# Autodesk Inventor assembly: B Idler
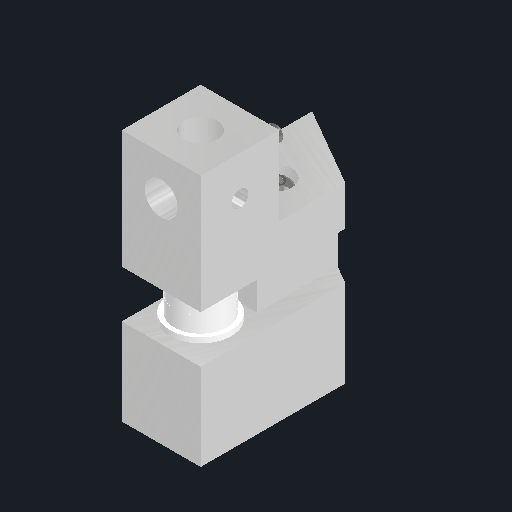
[picture p0: Inventor's stored thumbnail of the model, 512x512]
Saved by Autodesk Inventor 2025.1 (Build 291241020, 241B)
## iProperties
Created: 2025-05-09
Part Number: B Idler
Document SubType Name: Assembly
Designer: AdminForWorker
Title: B Idler
Author: AdminForWorker
## Documents named in this file (3)
- C:\Users\Joshua Eah\Documents\Voron 0.2\CAD\Master Assembly\B Idler.iam
- C:\Users\Joshua Eah\Documents\Voron 0.2\CAD\Master Assembly\Hardware\Hardware Assemblies\Hardware (10).iam
- C:\Users\Joshua Eah\Documents\Voron 0.2\CAD\Machined Parts\Idlers\B Idler\B Idler.ipt
## Components (2 placed, 2 different names)
1. Hardware (10):1 [sub-assembly] — Insert:1
2. B Idler:1 — Insert:1
## Relationships (1: Insert 1)
- Insert:1: Hardware (10):1 ↔ B Idler:1
